# Autodesk Inventor assembly: -ZPanel
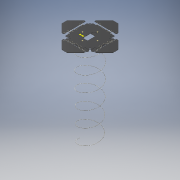
[picture p0: Inventor's stored thumbnail of the model, 180x180]
Saved by Autodesk Inventor 2018 (Build 220112000, 112)
## iProperties
Created: 2018-11-03
Part Number: -ZPanel
Document SubType Name: Assembly
Designer: Bradley
Author: Bradley
## Documents named in this file (12)
- C:\Users\Bradley\Documents\GitHub\CougSat1-Hardware\CougSat1-RadioBoard\CADModel\Native\-ZPanel.iam
- C:\Users\Bradley\Documents\GitHub\CougSat1-Hardware\CougSat1-RadioBoard\CADModel\Native\-ZPanel_PCB.ipt
- C:\Users\Bradley\Documents\GitHub\CougSat1-Hardware\CougSat1-RadioBoard\CADModel\Native\-ZPanel_AntennaDeloyed.ipt
- C:\Users\Bradley\Documents\GitHub\CougSat1-Hardware\CougSat1-RadioBoard\CADModel\Native\-ZPanel_AntennaStored.ipt
- C:\Users\Bradley\Documents\GitHub\CougSat1-Hardware\CougSat1-RadioBoard\CADModel\Native\-ZPanel_PCBExtender.ipt
- C:\Users\Bradley\Documents\GitHub\CougSat1-Hardware\CougSat1-RadioBoard\CADModel\Native\-ZPanel_SpringLeft.ipt
- C:\Users\Bradley\Documents\GitHub\CougSat1-Hardware\CougSat1-RadioBoard\CADModel\Native\-ZPanel_SpringRight.ipt
- C:\Users\Bradley\Documents\GitHub\CougSat1-Hardware\CougSat1-RadioBoard\CADModel\Native\-ZPanel_SpringDeployed.ipt
- C:\Users\Bradley\Documents\GitHub\Resources\SupplierDocuments\04 - Connectors SMT\04-0001\04-0001.iam
- C:\Users\Bradley\Documents\GitHub\Resources\SupplierDocuments\04 - Connectors SMT\04-0008\04-0008.iam
- C:\Users\Bradley\Documents\GitHub\Resources\SupplierDocuments\25 - Resistor THT\25-15.0\25-15.0.ipt
- C:\Users\Bradley\Documents\GitHub\Resources\SupplierDocuments\04 - Connectors SMT\04-0009\04-0009.iam
## Components (51 placed, 11 different names)
1. 04-0001:1 [sub-assembly] — Mate:6, Mate:7, Flush:6
2. 04-0008:1 [sub-assembly] — Mate:5, Flush:7, Mate:8
3. 04-0009:1 [sub-assembly] — Insert:10
4. 04-0009:2 [sub-assembly] — Insert:11
5. 04-0009:3 [sub-assembly] — Insert:12
6. 04-0009:4 [sub-assembly] — Insert:13
7. 25-15.0:1 — Insert:4, Insert:5
8. 25-15.0:2 — Insert:2, Insert:3
9. -ZPanel_AntennaDeloyed:1 — Mate:11, Mate:12, Mate:1
10. -ZPanel_AntennaStored:1 — Mate:9, Mate:10, Mate:2
11. -ZPanel_PCB:1 — Mate:1, Mate:2, Mate:5, Mate:6, Insert:2, Insert:3, Insert:4, Insert:5, Mate:13, Mate:14, Flush:8, Flush:9, Flush:10, Flush:11, Flush:12, Flush:13, Flush:14, Flush:15, Flush:16, Flush:17, Mate:20, Insert:10, Insert:11, Insert:12, Insert:13
12. -ZPanel_PCBExtender:1 — Mate:13, Mate:14, Flush:16
13. -ZPanel_SpringLeft:1 — Flush:8, Mate:15, Flush:9, Insert:6
14. -ZPanel_SpringRight:1 — Flush:12, Flush:13, Mate:17, Insert:9
15. -ZPanel_SpringRight:2 — Mate:18, Flush:14, Flush:15, Insert:8
16. -ZPanel_SpringLeft:2 — Mate:16, Flush:10, Flush:11, Insert:7
17. -ZPanel_PCBExtender:2
18. -ZPanel_SpringLeft:3
19. -ZPanel_SpringRight:3
20. -ZPanel_SpringRight:4
21. -ZPanel_SpringLeft:4
22. -ZPanel_PCBExtender:3
23. -ZPanel_SpringLeft:5
24. -ZPanel_SpringRight:5
25. -ZPanel_SpringRight:6
26. -ZPanel_SpringLeft:6
27. -ZPanel_PCBExtender:4
28. -ZPanel_SpringLeft:7
29. -ZPanel_SpringRight:7
30. -ZPanel_SpringRight:8
31. -ZPanel_SpringLeft:8
32. -ZPanel_SpringDeployed:1 — Insert:6
33. -ZPanel_SpringDeployed:2 — Insert:7
34. -ZPanel_SpringDeployed:3 — Insert:8
35. -ZPanel_SpringDeployed:4 — Insert:9
36. -ZPanel_PCBExtender:5 — Mate:19, Flush:17, Mate:20
37. -ZPanel_SpringDeployed:5
38. -ZPanel_SpringDeployed:6
39. -ZPanel_SpringDeployed:7
40. -ZPanel_SpringDeployed:8
41. -ZPanel_PCBExtender:6
42. -ZPanel_SpringDeployed:9
43. -ZPanel_SpringDeployed:10
44. -ZPanel_SpringDeployed:11
45. -ZPanel_SpringDeployed:12
46. -ZPanel_PCBExtender:7
47. -ZPanel_SpringDeployed:13
48. -ZPanel_SpringDeployed:14
49. -ZPanel_SpringDeployed:15
50. -ZPanel_SpringDeployed:16
51. -ZPanel_PCBExtender:8
## Component patterns: (4 elements, first: -ZPanel_PCBExtender:1 + -ZPanel_SpringLeft:1 + -ZPanel_SpringRight:1 + -ZPanel_SpringRight:2 + -ZPanel_SpringLeft:2), (4 elements, first: -ZPanel_SpringDeployed:1 + -ZPanel_SpringDeployed:2 + -ZPanel_SpringDeployed:3 + -ZPanel_SpringDeployed:4 + -ZPanel_PCBExtender:5)
## Relationships (42: Mate 18, Flush 12, Insert 12)
- Mate:11: -ZPanel_AntennaDeloyed:1
- Mate:12: -ZPanel_AntennaDeloyed:1
- Mate:1 (0.2794 mm): -ZPanel_AntennaDeloyed:1 ↔ -ZPanel_PCB:1
- Mate:9: -ZPanel_AntennaStored:1
- Mate:10: -ZPanel_AntennaStored:1
- Mate:2 (0.2794 mm): -ZPanel_AntennaStored:1 ↔ -ZPanel_PCB:1
- Mate:5: 04-0008:1 ↔ -ZPanel_PCB:1
- Mate:6: 04-0001:1 ↔ -ZPanel_PCB:1
- Mate:7 (-14 mm): 04-0001:1
- Flush:6 (20 mm): 04-0001:1
- Flush:7 (15 mm): 04-0008:1
- Mate:8 (-22 mm): 04-0008:1
- Insert:2 (-1.5 mm): 25-15.0:2 ↔ -ZPanel_PCB:1
- Insert:3 (-1.5 mm): 25-15.0:2 ↔ -ZPanel_PCB:1
- Insert:4 (-1.5 mm): 25-15.0:1 ↔ -ZPanel_PCB:1
- Insert:5 (-1.5 mm): 25-15.0:1 ↔ -ZPanel_PCB:1
- Mate:13 (-4 mm): -ZPanel_PCB:1 ↔ -ZPanel_PCBExtender:1
- Mate:14: -ZPanel_PCB:1 ↔ -ZPanel_PCBExtender:1
- Flush:8 (2 mm): -ZPanel_PCB:1 ↔ -ZPanel_SpringLeft:1
- Mate:15 (-24 mm): -ZPanel_SpringLeft:1
- Flush:9: -ZPanel_PCB:1 ↔ -ZPanel_SpringLeft:1
- Mate:16 (-13 mm): -ZPanel_SpringLeft:2
- Flush:10: -ZPanel_PCB:1 ↔ -ZPanel_SpringLeft:2
- Flush:11 (2 mm): -ZPanel_PCB:1 ↔ -ZPanel_SpringLeft:2
- Flush:12: -ZPanel_PCB:1 ↔ -ZPanel_SpringRight:1
- Flush:13 (2 mm): -ZPanel_PCB:1 ↔ -ZPanel_SpringRight:1
- Mate:17 (24 mm): -ZPanel_SpringRight:1
- Mate:18 (13 mm): -ZPanel_SpringRight:2
- Flush:14 (2 mm): -ZPanel_PCB:1 ↔ -ZPanel_SpringRight:2
- Flush:15: -ZPanel_PCB:1 ↔ -ZPanel_SpringRight:2
- Flush:16: -ZPanel_PCB:1 ↔ -ZPanel_PCBExtender:1
- Insert:6: -ZPanel_SpringLeft:1 ↔ -ZPanel_SpringDeployed:1
- Insert:7: -ZPanel_SpringLeft:2 ↔ -ZPanel_SpringDeployed:2
- Insert:8: -ZPanel_SpringRight:2 ↔ -ZPanel_SpringDeployed:3
- Insert:9: -ZPanel_SpringRight:1 ↔ -ZPanel_SpringDeployed:4
- Mate:19: -ZPanel_PCBExtender:5
- Flush:17: -ZPanel_PCB:1 ↔ -ZPanel_PCBExtender:5
- Mate:20 (4.736 mm): -ZPanel_PCB:1 ↔ -ZPanel_PCBExtender:5
- Insert:10: 04-0009:1 ↔ -ZPanel_PCB:1
- Insert:11: 04-0009:2 ↔ -ZPanel_PCB:1
- Insert:12: 04-0009:3 ↔ -ZPanel_PCB:1
- Insert:13: 04-0009:4 ↔ -ZPanel_PCB:1
